# Autodesk Inventor assembly: dtmotorgearsdeadaxle
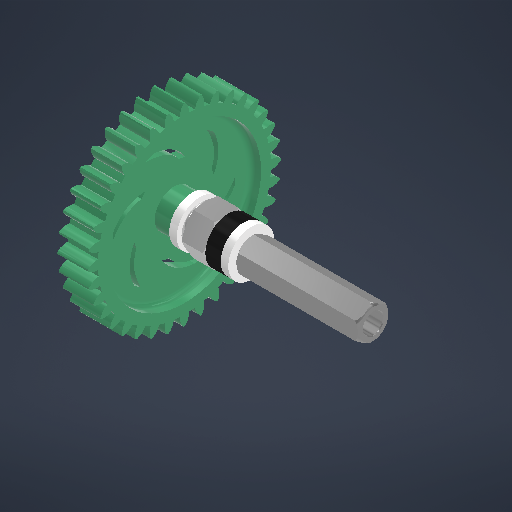
[picture p0: Inventor's stored thumbnail of the model, 512x512]
Saved by Autodesk Inventor 2026.1 (Build 301233000, 233)
## iProperties
Created: 2025-08-03
Part Number: dtmotorgearsdeadaxle
Document SubType Name: Assembly
Designer: roejo
Author: roejo
## Documents named in this file (9)
- C:\Users\roejo\OneDrive\Documents\3284b-cad-2025\Robots\Highlander\SubAssemblies\dtmotorgearsdeadaxle.iam
- C:\Users\roejo\OneDrive\Documents\3284b-cad-2025\Library\VEX-CAD-Inventor-1.4.2\Motion\Gears\LS 36T Gear.ipt
- C:\Users\roejo\OneDrive\Documents\3284b-cad-2025\Library\VEX-CAD-Inventor-1.4.2\Motion\Spacers\Washer Teflon\TWasher .375 OD x .06250.ipt
- C:\Users\roejo\OneDrive\Documents\3284b-cad-2025\Library\VEX-CAD-Inventor-1.4.2\Motion\Spacers\Washer Teflon.ipt
- C:\Users\roejo\OneDrive\Documents\3284b-cad-2025\Library\VEX-CAD-Inventor-1.4.2\Motion\Spacers\Spacer Nylon .375 OD.ipt
- C:\Users\roejo\OneDrive\Documents\3284b-cad-2025\Library\VEX-CAD-Inventor-1.4.2\Motion\Spacers\Spacer Nylon .375 OD\NSpacer .375 OD x .125.ipt
- C:\Users\roejo\OneDrive\Documents\3284b-cad-2025\Library\VEX-CAD-Inventor-1.4.2\Structure\Hardware\alu_nylock.ipt
- C:\Users\roejo\OneDrive\Documents\3284b-cad-2025\Library\VEX-CAD-Inventor-1.4.2\Structure\Standoff\Standoff 1.00.ipt
- C:\Users\roejo\OneDrive\Documents\3284b-cad-2025\Library\VEX-CAD-Inventor-1.4.2\Structure\Standoff.ipt
## Components (7 placed, 5 different names)
1. LS 36T Gear:1 — Insert:1, Insert:2
2. TWasher .375 OD x .06250:1 — Insert:1
3. TWasher .375 OD x .06250:2 — Insert:2, Insert:3
4. alu_nylock:1 — Insert:3, Insert:4
5. Standoff 1.00:1 — Insert:6
6. NSpacer .375 OD x .125:1 — Insert:4, Insert:5
7. TWasher .375 OD x .06250:4 — Insert:5, Insert:6
## Relationships (6: Insert 6)
- Insert:1: LS 36T Gear:1 ↔ TWasher .375 OD x .06250:1
- Insert:2: LS 36T Gear:1 ↔ TWasher .375 OD x .06250:2
- Insert:3: TWasher .375 OD x .06250:2 ↔ alu_nylock:1
- Insert:4: alu_nylock:1 ↔ NSpacer .375 OD x .125:1
- Insert:5: NSpacer .375 OD x .125:1 ↔ TWasher .375 OD x .06250:4
- Insert:6: Standoff 1.00:1 ↔ TWasher .375 OD x .06250:4
